# Autodesk Inventor assembly: 313-01
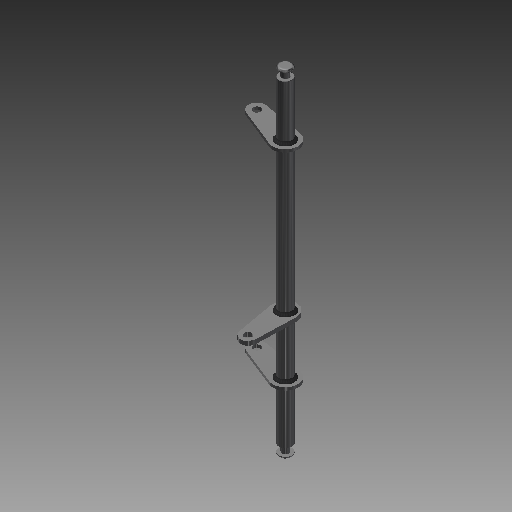
[picture p0: Inventor's stored thumbnail of the model, 512x512]
Saved by Autodesk Inventor 2019 (Build 230136000, 136)
## iProperties
Company: Autodesk Inc.
Created: 2007-10-25
Part Number: 313-01
Description: PIVOT LINK WELDMENT
Document SubType Name: Weldment
Designer: Autodesk Inc.
Weld Material: Welded Steel Mild (Black-Flat)
Mass: 742.298 g
Surface Area: 352.97 cm^2
Volume: 94.5583 cm^3
Density: 7.85016 g/cm^3
Component Category: Lower Component
Author: Inventor
## Documents named in this file (4)
- C:\TEMP\Car Seat\Workspace\Rear Pivot Link Weldment_MIR.iam
- C:\TEMP\Car Seat\Workspace\HOR Support Bar.ipt
- C:\TEMP\Car Seat\Workspace\Rear Pivot Plate B.ipt
- C:\TEMP\Car Seat\Workspace\Rear Pivot Plate A.ipt
## Components (4 placed, 3 different names)
1. Rear Pivot Plate A:2 — Flush:2, Mate:1
2. Rear Pivot Plate A:1 — Flush:1, Mate:2
3. HOR Support Bar:1 — Flush:2, Flush:1, Mate:2, Mate:1, Mate:4
4. Rear Pivot Plate B:1 — Mate:4
## Relationships (8: Flush 4, Mate 3, Angle 1)
- [Flush]: Rear Pivot Plate A:2 ↔ Rear Pivot Plate A:1
- Flush:2 (-64.5 mm): Rear Pivot Plate A:2 ↔ HOR Support Bar:1
- Flush:1 (64.5 mm): Rear Pivot Plate A:1 ↔ HOR Support Bar:1
- Mate:2: Rear Pivot Plate A:1 ↔ HOR Support Bar:1
- Mate:1: Rear Pivot Plate A:2 ↔ HOR Support Bar:1
- Mate:4: HOR Support Bar:1 ↔ Rear Pivot Plate B:1
- [Angle] (250 deg): Rear Pivot Plate A:2 ↔ Rear Pivot Plate B:1
- [Flush] (54.165 mm): HOR Support Bar:1 ↔ Rear Pivot Plate B:1
